# Autodesk Inventor assembly: Assembly1
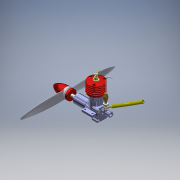
[picture p0: Inventor's stored thumbnail of the model, 180x180]
Saved by Autodesk Inventor 2018.1 (Build 221171000, 171)
## iProperties
Created: 2013-08-27
Part Number: Assembly1
Document SubType Name: Assembly
Designer: Konstantin
Author: Konstantin
## Documents named in this file (21)
- C:\Users\Konstantin\Desktop\Inventor To Do\MK-16\mk-16.iam
- C:\Users\Konstantin\Desktop\Inventor To Do\MK-16\main_body.ipt
- C:\Users\Konstantin\Desktop\Inventor To Do\MK-16\cam.ipt
- C:\Users\Konstantin\Desktop\Inventor To Do\MK-16\cover.ipt
- C:\Users\Konstantin\Desktop\Inventor To Do\MK-16\cylinder.ipt
- C:\Users\Konstantin\Desktop\Inventor To Do\MK-16\piston.ipt
- C:\Users\Konstantin\Desktop\Inventor To Do\MK-16\pin.ipt
- C:\Users\Konstantin\Desktop\Inventor To Do\MK-16\throttle.ipt
- C:\Users\Konstantin\Desktop\Inventor To Do\MK-16\stud.ipt
- C:\Users\Konstantin\Desktop\Inventor To Do\MK-16\compression_ratio.ipt
- C:\Users\Konstantin\Desktop\Inventor To Do\MK-16\fuel_inlet.ipt
- C:\Users\Konstantin\Desktop\Inventor To Do\MK-16\rod.ipt
- C:\Users\Konstantin\Desktop\Inventor To Do\MK-16\shaft.ipt
- C:\Users\Konstantin\Desktop\Inventor To Do\MK-16\Bearing 1006095 GOST 831-75.ipt
- C:\Users\Konstantin\Desktop\Inventor To Do\MK-16\ISO 7045 - M2,5 x 5 - 4.8 - HDIN EN ISO.ipt
- C:\Users\Konstantin\Desktop\Inventor To Do\MK-16\ISO 7045 - M2,5 x 10 - 4.8 - HDIN EN ISO.ipt
- C:\Users\Konstantin\Desktop\Inventor To Do\MK-16\pad.ipt
- C:\Users\Konstantin\Desktop\Inventor To Do\MK-16\propeller.ipt
- C:\Users\Konstantin\Desktop\Inventor To Do\MK-16\washer.ipt
- C:\Users\Konstantin\Desktop\Inventor To Do\MK-16\nose-over.ipt
- C:\Users\Konstantin\Desktop\Inventor To Do\MK-16\hose.ipt
## Components (26 placed, 20 different names)
1. main_body:1 — Mate:1, Mate:2, Mate:3, Mate:4, Mate:17, Mate:18, Mate:41, Mate:45, Mate:53, Mate:59
2. cylinder:1 — Mate:1, Mate:2, Mate:8, Mate:14, Mate:42, Mate:43, Mate:44, Mate:45, Mate:46, Mate:47, Mate:48, Flush:1
3. cover:1 — Mate:3, Mate:4, Mate:5, Mate:6, Mate:9, Mate:11, Mate:49, Mate:50, Mate:51, Mate:52, Mate:53, Mate:54, Mate:55, Mate:56, Mate:57
4. cam:1 — Mate:5, Mate:6, Mate:19
5. piston:1 — Mate:7, Tangent:1, Mate:8, Mate:16
6. pin:1 — Mate:7, Tangent:1, Mate:15
7. throttle:1 — Mate:13
8. stud:1 — Mate:9, Mate:10, Mate:12, Mate:13
9. compression_ratio:1 — Mate:14, Flush:1
10. fuel_inlet:1 — Mate:10, Mate:11, Mate:12, Mate:68, Mate:69
11. rod:1 — Mate:15, Mate:16, Mate:20
12. shaft:1 — Mate:17, Mate:18, Mate:19, Mate:20, Mate:40, Mate:58, Mate:60, Mate:61, Mate:62, Mate:63, Mate:64, Mate:66, Mate:67
13. Bearing 6000 GOST 831-75 1006095:1 — Mate:40, Mate:41
14. DIN EN ISO 7045 H M2,5 x 5 - 4.8 - H:1 — Mate:49, Mate:55
15. DIN EN ISO 7045 H M2,5 x 5 - 4.8 - H:2 — Mate:52, Mate:54
16. DIN EN ISO 7045 H M2,5 x 5 - 4.8 - H:3 — Mate:51, Mate:56
17. DIN EN ISO 7045 H M2,5 x 5 - 4.8 - H:4 — Mate:50, Mate:57
18. DIN EN ISO 7045 H M2,5 x 10 - 4.8 - H:1 — Mate:43, Mate:47
19. DIN EN ISO 7045 H M2,5 x 10 - 4.8 - H:2 — Mate:42, Mate:46
20. DIN EN ISO 7045 H M2,5 x 10 - 4.8 - H:3 — Mate:44, Mate:48
21. Bearing 6000 GOST 831-75 1006095:2 — Mate:58, Mate:59
22. pad:1 — Mate:60, Mate:61
23. propeller:1 — Mate:62, Mate:63, Mate:65
24. washer:1 — Mate:64, Mate:65
25. nose-over:1 — Mate:66, Mate:67
26. hose:1 — Mate:68, Mate:69
## Relationships (52: Mate 50, Tangent 1, Flush 1)
- Mate:1: main_body:1 ↔ cylinder:1
- Mate:2: main_body:1 ↔ cylinder:1
- Mate:3: main_body:1 ↔ cover:1
- Mate:4: main_body:1 ↔ cover:1
- Mate:5: cover:1 ↔ cam:1
- Mate:6: cover:1 ↔ cam:1
- Mate:7: piston:1 ↔ pin:1
- Tangent:1: piston:1 ↔ pin:1
- Mate:8: cylinder:1 ↔ piston:1
- Mate:9: cover:1 ↔ stud:1
- Mate:10: stud:1 ↔ fuel_inlet:1
- Mate:11: cover:1 ↔ fuel_inlet:1
- Mate:12: stud:1 ↔ fuel_inlet:1
- Mate:13: throttle:1 ↔ stud:1
- Mate:14: cylinder:1 ↔ compression_ratio:1
- Mate:15: pin:1 ↔ rod:1
- Mate:16 (1 mm): piston:1 ↔ rod:1
- Mate:17: main_body:1 ↔ shaft:1
- Mate:18: main_body:1 ↔ shaft:1
- Mate:19: cam:1 ↔ shaft:1
- Mate:20: rod:1 ↔ shaft:1
- Mate:40: shaft:1 ↔ Bearing 6000 GOST 831-75 1006095:1
- Mate:41: main_body:1 ↔ Bearing 6000 GOST 831-75 1006095:1
- Mate:42: cylinder:1 ↔ DIN EN ISO 7045 H M2,5 x 10 - 4.8 - H:2
- Mate:43: cylinder:1 ↔ DIN EN ISO 7045 H M2,5 x 10 - 4.8 - H:1
- Mate:44: cylinder:1 ↔ DIN EN ISO 7045 H M2,5 x 10 - 4.8 - H:3
- Mate:45: main_body:1 ↔ cylinder:1
- Mate:46: cylinder:1 ↔ DIN EN ISO 7045 H M2,5 x 10 - 4.8 - H:2
- Mate:47: cylinder:1 ↔ DIN EN ISO 7045 H M2,5 x 10 - 4.8 - H:1
- Mate:48: cylinder:1 ↔ DIN EN ISO 7045 H M2,5 x 10 - 4.8 - H:3
- Flush:1: cylinder:1 ↔ compression_ratio:1
- Mate:49: cover:1 ↔ DIN EN ISO 7045 H M2,5 x 5 - 4.8 - H:1
- Mate:50: cover:1 ↔ DIN EN ISO 7045 H M2,5 x 5 - 4.8 - H:4
- Mate:51: cover:1 ↔ DIN EN ISO 7045 H M2,5 x 5 - 4.8 - H:3
- Mate:52: cover:1 ↔ DIN EN ISO 7045 H M2,5 x 5 - 4.8 - H:2
- Mate:53: main_body:1 ↔ cover:1
- Mate:54: cover:1 ↔ DIN EN ISO 7045 H M2,5 x 5 - 4.8 - H:2
- Mate:55: cover:1 ↔ DIN EN ISO 7045 H M2,5 x 5 - 4.8 - H:1
- Mate:56: cover:1 ↔ DIN EN ISO 7045 H M2,5 x 5 - 4.8 - H:3
- Mate:57: cover:1 ↔ DIN EN ISO 7045 H M2,5 x 5 - 4.8 - H:4
- Mate:58: shaft:1 ↔ Bearing 6000 GOST 831-75 1006095:2
- Mate:59: main_body:1 ↔ Bearing 6000 GOST 831-75 1006095:2
- Mate:60: shaft:1 ↔ pad:1
- Mate:61: shaft:1 ↔ pad:1
- Mate:62: shaft:1 ↔ propeller:1
- Mate:63: shaft:1 ↔ propeller:1
- Mate:64: shaft:1 ↔ washer:1
- Mate:65: propeller:1 ↔ washer:1
- Mate:66: shaft:1 ↔ nose-over:1
- Mate:67: shaft:1 ↔ nose-over:1
- Mate:68: fuel_inlet:1 ↔ hose:1
- Mate:69 (-3 mm): fuel_inlet:1 ↔ hose:1
